# Autodesk Inventor assembly: coupler extenison arm motor+ servo mount
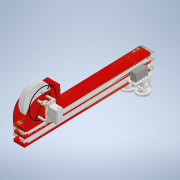
[picture p0: Inventor's stored thumbnail of the model, 180x180]
Saved by Autodesk Inventor 2020 (Build 240168000, 168)
## iProperties
Created: 2019-12-15
Part Number: coupler extenison arm motor+ servo mount
Document SubType Name: Assembly
Designer: ball
Author: ball
## Documents named in this file (13)
- D:\FTC8863\2019 Robot\Delivery\extension arm\coupler extenison arm motor+ servo mount.iam
- D:\FTC8863\2019 Robot\Delivery\extension arm\Coupler extension arm motor.ipt
- D:\FTC8863\2019 Robot\Delivery\extension arm\Coupler extension arm short.ipt
- D:\FTC8863\Misumi\SAR340\SAR340 offset 10 mm.iam
- D:\FTC8863\RevRobotics\REV-41-1368 pulley.ipt
- D:\FTC8863\2019 Robot\Delivery\plastic pulley deep u.ipt
- D:\FTC8863\2019 Robot\Delivery\extension arm\extension arm top.iam
- D:\FTC8863\2019 Robot\Collection\servo block assembly.iam
- D:\FTC8863\2019 Robot\Delivery\extension arm\Coupler extension arm short edited holes for servo.ipt
- D:\FTC8863\Actobotics\615 parts\615190.ipt
- D:\FTC8863\Actobotics\545 parts\545364 assembly.ipt
- D:\FTC8863\2019 Robot\Delivery\extension arm\standoff for gripper servo.ipt
- D:\FTC8863\2019 Robot\Delivery\extension arm\Servo mount + servo.iam
## Components (17 placed, 12 different names)
1. Coupler extension arm motor:1 — Mate:3, Flush:4, Flush:5, Flush:6, Flush:7, Mate:5, Mate:6, Mate:7, Flush:8, Flush:10, Flush:11
2. Coupler extension arm short:1 — Mate:3, Flush:4, Flush:5, Mate:4, Mate:8, Mate:9, Mate:10, Mate:11, Mate:12, Flush:9
3. SAR340 offset 10 mm:1 [sub-assembly] — Mate:4, Flush:6, Flush:7, Mate:13
4. REV-41-1368 pulley:1 — Mate:5, Mate:6
5. REV-41-1368 pulley:2 — Mate:7, Flush:8
6. REV-41-1368 pulley:3 — Mate:9, Mate:10
7. REV-41-1368 pulley:4 — Mate:8, Mate:11
8. plastic pulley deep u:1 — Mate:12, Flush:9
9. extension arm top:1 [sub-assembly] — Mate:13, Flush:10, Flush:11, Mate:15, Flush:14, Flush:15
10. Coupler extension arm motor:2 — Flush:12, Flush:13, Mate:14, Mate:15, Flush:14, Flush:15
11. Coupler extension arm short edited holes for servo:1 — Flush:12, Flush:13, Mate:14, Mate:16, Mate:17, Mate:25, Mate:26, Mate:27, Mate:32, Mate:33, Mate:34
12. servo block assembly:1 [sub-assembly] — Mate:16, Mate:17, Mate:28, Mate:29, Mate:30, Mate:31
13. 615190:1 — Mate:35, Mate:36, Mate:37
14. 615190:2 — Mate:29, Mate:30, Mate:31
15. 545364 assembly:1 — Mate:32, Mate:33, Mate:34, Mate:35, Mate:36, Mate:37
16. standoff for gripper servo:1 — Mate:25, Mate:26, Mate:27, Mate:28
17. Servo mount + servo:1 [sub-assembly]
## Relationships (44: Mate 28, Flush 15, Angle 1)
- [Flush]: Coupler extension arm motor:1 ↔ Servo mount + servo:1
- [Flush]: Coupler extension arm motor:1 ↔ Servo mount + servo:1
- [Flush]: Coupler extension arm motor:1 ↔ Servo mount + servo:1
- [Angle] (0 deg): Coupler extension arm motor:1 ↔ Servo mount + servo:1
- Mate:3: Coupler extension arm motor:1 ↔ Coupler extension arm short:1
- Flush:4: Coupler extension arm motor:1 ↔ Coupler extension arm short:1
- Flush:5: Coupler extension arm motor:1 ↔ Coupler extension arm short:1
- Mate:4: Coupler extension arm short:1 ↔ SAR340 offset 10 mm:1
- Flush:6: Coupler extension arm motor:1 ↔ SAR340 offset 10 mm:1
- Flush:7: Coupler extension arm motor:1 ↔ SAR340 offset 10 mm:1
- Mate:5: Coupler extension arm motor:1 ↔ REV-41-1368 pulley:1
- Mate:6: Coupler extension arm motor:1 ↔ REV-41-1368 pulley:1
- Mate:7: Coupler extension arm motor:1 ↔ REV-41-1368 pulley:2
- Flush:8: Coupler extension arm motor:1 ↔ REV-41-1368 pulley:2
- Mate:8: Coupler extension arm short:1 ↔ REV-41-1368 pulley:4
- Mate:9: Coupler extension arm short:1 ↔ REV-41-1368 pulley:3
- Mate:10: Coupler extension arm short:1 ↔ REV-41-1368 pulley:3
- Mate:11: Coupler extension arm short:1 ↔ REV-41-1368 pulley:4
- Mate:12: Coupler extension arm short:1 ↔ plastic pulley deep u:1
- Flush:9: Coupler extension arm short:1 ↔ plastic pulley deep u:1
- Mate:13: SAR340 offset 10 mm:1 ↔ extension arm top:1
- Flush:10: Coupler extension arm motor:1 ↔ extension arm top:1
- Flush:11: Coupler extension arm motor:1 ↔ extension arm top:1
- Flush:12: Coupler extension arm motor:2 ↔ Coupler extension arm short edited holes for servo:1
- Flush:13: Coupler extension arm motor:2 ↔ Coupler extension arm short edited holes for servo:1
- Mate:14: Coupler extension arm motor:2 ↔ Coupler extension arm short edited holes for servo:1
- Mate:15: extension arm top:1 ↔ Coupler extension arm motor:2
- Flush:14: extension arm top:1 ↔ Coupler extension arm motor:2
- Flush:15: extension arm top:1 ↔ Coupler extension arm motor:2
- Mate:16: Coupler extension arm short edited holes for servo:1 ↔ servo block assembly:1
- Mate:17: Coupler extension arm short edited holes for servo:1 ↔ servo block assembly:1
- Mate:25: Coupler extension arm short edited holes for servo:1 ↔ standoff for gripper servo:1
- Mate:26: Coupler extension arm short edited holes for servo:1 ↔ standoff for gripper servo:1
- Mate:27: Coupler extension arm short edited holes for servo:1 ↔ standoff for gripper servo:1
- Mate:28: servo block assembly:1 ↔ standoff for gripper servo:1
- Mate:29: servo block assembly:1 ↔ 615190:2
- Mate:30: servo block assembly:1 ↔ 615190:2
- Mate:31: servo block assembly:1 ↔ 615190:2
- Mate:32: Coupler extension arm short edited holes for servo:1 ↔ 545364 assembly:1
- Mate:33: Coupler extension arm short edited holes for servo:1 ↔ 545364 assembly:1
- Mate:34: Coupler extension arm short edited holes for servo:1 ↔ 545364 assembly:1
- Mate:35: 615190:1 ↔ 545364 assembly:1
- Mate:36: 615190:1 ↔ 545364 assembly:1
- Mate:37: 615190:1 ↔ 545364 assembly:1
